# Autodesk Inventor assembly: atmega
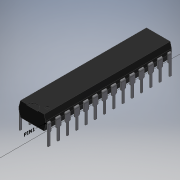
[picture p0: Inventor's stored thumbnail of the model, 180x180]
Saved by Autodesk Inventor 2018 (Build 220112000, 112)
## iProperties
Created: 2017-04-13
Part Number: atmega
Document SubType Name: Assembly
Designer: kampe_000
atmegaPinDistance: 2,540 mm
Author: kampe_000
## Documents named in this file (5)
- D:\Kod\stepCounter\CAD\Inventor Project\assembly\atmega.iam
- D:\Kod\stepCounter\CAD\Inventor Project\parts\atmega_mold.ipt
- D:\Kod\stepCounter\CAD\Inventor Project\parts\atmega_pin.ipt
- D:\Kod\stepCounter\CAD\Inventor Project\parts\atmega_pin-end.ipt
- D:\Kod\stepCounter\CAD\Inventor Project\parts\atmega_pin-end_MIR.ipt
## Components (15 placed, 4 different names)
1. atmega_mold:1 — Mate:1, Mate:2, Mate:3, Flush:1, Mate:4, Mate:5, Flush:2, Mate:6
2. atmega_pin-end:1 — Mate:4, Mate:5, Flush:2
3. atmega_pin-end_MIR:1
4. atmega_pin:1 — Mate:2, Mate:3, Flush:1
5. atmega_pin:2
6. atmega_pin:3
7. atmega_pin:4
8. atmega_pin:5
9. atmega_pin:6
10. atmega_pin:7
11. atmega_pin:8
12. atmega_pin:9
13. atmega_pin:10
14. atmega_pin:11
15. atmega_pin:12
## Component patterns: (12 elements, first: atmega_pin:1)
## Relationships (8: Mate 6, Flush 2)
- Mate:1: atmega_mold:1
- Mate:2: atmega_mold:1 ↔ atmega_pin:1
- Mate:3: atmega_mold:1 ↔ atmega_pin:1
- Flush:1: atmega_mold:1 ↔ atmega_pin:1
- Mate:4: atmega_mold:1 ↔ atmega_pin-end:1
- Mate:5: atmega_mold:1 ↔ atmega_pin-end:1
- Flush:2: atmega_mold:1 ↔ atmega_pin-end:1
- Mate:6: atmega_mold:1
## Named parameters: atmegaPinDistance = 2.54 mm
